# Autodesk Inventor assembly: EV-ADF4360
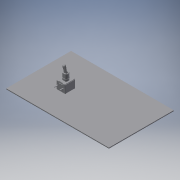
[picture p0: Inventor's stored thumbnail of the model, 180x180]
Saved by Autodesk Inventor 2018 (Build 220112000, 112)
## iProperties
Created: 2018-04-06
Part Number: EV-ADF4360
Document SubType Name: Assembly
Designer: bbramman
Author: bbramman
## Documents named in this file (3)
- C:\Users\bbramman\OneDrive\Documents\Trapped Ion Research (Grad)\Electronics\pll-evalboard-synthesizer\Box CAD\EV-ADF4360.iam
- C:\Users\bbramman\OneDrive\Documents\Trapped Ion Research (Grad)\Electronics\pll-evalboard-synthesizer\Box CAD\95x60mm-PCB.ipt
- C:\Users\bbramman\OneDrive\Documents\Trapped Ion Research (Grad)\Electronics\pll-evalboard-synthesizer\Box CAD\Switch.iam
## Components (2 placed, 2 different names)
1. 95x60mm-PCB:1 — Mate:1
2. Switch:1 [sub-assembly] — Mate:1
## Relationships (1: Mate 1)
- Mate:1: 95x60mm-PCB:1 ↔ Switch:1
